# Autodesk Inventor assembly: 감속기어1
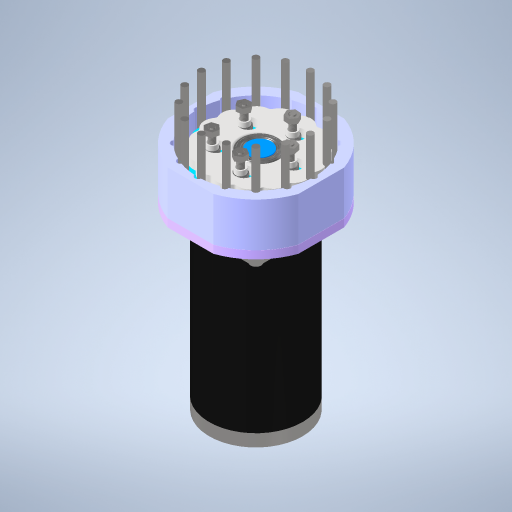
[picture p0: Inventor's stored thumbnail of the model, 512x512]
Saved by Autodesk Inventor 2023 (Build 270158000, 158)
## iProperties
Created: 2022-06-20
Part Number: 감속기어1
Document SubType Name: Assembly
Designer: user
Author: user
## Documents named in this file (19)
- C:\Users\user\Desktop\Baymax-main\설계\출력 부품\감속기어1.iam
- C:\Users\user\Desktop\Baymax-main\설계\범용 부품\베어링 6810.ipt
- C:\Users\user\Desktop\Baymax-main\설계\범용 부품\M4 16mm 십자나사.ipt
- C:\Users\user\Desktop\Baymax-main\설계\범용 부품\M4 너트.ipt
- C:\Users\user\Desktop\Baymax-main\설계\범용 부품\중형 모터 MB60080-2430 DC24V.ipt
- C:\Users\user\Desktop\Baymax-main\설계\출력 부품\감속기어1 - 기어 하우징.ipt
- C:\Users\user\Desktop\Baymax-main\설계\출력 부품\감속기어1 - 사이클로이드 기어.ipt
- C:\Users\user\Desktop\Baymax-main\설계\출력 부품\감속기어1 - 사이클로이드 회전축.ipt
- C:\Users\user\Desktop\Baymax-main\설계\범용 부품\M4 30mm 십자나사.ipt
- C:\Users\user\Desktop\Baymax-main\설계\출력 부품\감속기어1 - 축.ipt
- C:\Users\user\Desktop\Baymax-main\설계\범용 부품\베어링 6802.ipt
- C:\Users\user\Desktop\Baymax-main\설계\범용 부품\베어링 MR84ZZ.ipt
- C:\Users\user\Desktop\Baymax-main\설계\출력 부품\감속기어1 - 하우징 커버.ipt
- C:\Users\user\Desktop\Baymax-main\설계\범용 부품\4파이 20mm 핀.ipt
- C:\Users\user\Desktop\Baymax-main\설계\출력 부품\감속기어1 - 상단 편심축.ipt
- C:\Users\user\Desktop\Baymax-main\설계\출력 부품\감속기어1 - 4파이 4mm와셔.ipt
- C:\Users\user\Desktop\Baymax-main\설계\출력 부품\감속기어1 - 4파이 3mm와셔.ipt
- C:\Users\user\Desktop\Baymax-main\설계\출력 부품\감속기어1 - 회전축 상단.ipt
- C:\Users\user\Desktop\Baymax-main\설계\출력 부품\감속기어1 - 하우징 상단 커버.ipt
## Components (72 placed, 18 different names)
1. 베어링 6810:1 — 회전:5, 삽입:2
2. 중형 모터 MB60080-2430 DC24V:1 — 강체:1, 회전:7, 회전:8, 회전:9, 삽입:5, 회전:14
3. 감속기어1 - 기어 하우징:1 — 회전:1, 회전:2, 회전:3, 회전:4, 회전:5, 회전:13, 회전:15, 메이트:16
4. 감속기어1 - 사이클로이드 기어:1 — 삽입:4
5. 감속기어1 - 사이클로이드 회전축:1 — 강체:2, 강체:3, 회전:10, 회전:11, 회전:12, 삽입:2, 메이트:1, 메이트:2, 메이트:3, 메이트:4, 메이트:5, 메이트:6, 메이트:7, 메이트:8, 메이트:9, 메이트:10
6. M4 너트:1 — 회전:4
7. M4 너트:2 — 회전:3
8. M4 너트:3 — 회전:2
9. M4 너트:4 — 회전:1
10. M4 16mm 십자나사:1 — 회전:7
11. M4 16mm 십자나사:2 — 강체:1
12. M4 16mm 십자나사:3 — 회전:9
13. M4 16mm 십자나사:4 — 회전:8
14. M4 30mm 십자나사:1 — 회전:10
15. M4 30mm 십자나사:2 — 강체:2
16. M4 30mm 십자나사:3 — 강체:3
17. M4 30mm 십자나사:4 — 회전:12
18. M4 30mm 십자나사:5 — 회전:11
19. 감속기어1 - 축:1 — 삽입:3, 삽입:5, 회전:16
20. 베어링 6802:1 — 삽입:3, 삽입:4
21. 베어링 MR84ZZ:1 — 메이트:11
22. M4 너트:6 — 메이트:3, 메이트:4, 메이트:11
23. M4 너트:7 — 메이트:7, 메이트:8, 메이트:13
24. M4 너트:8 — 메이트:9, 메이트:10, 메이트:15
25. M4 너트:9 — 메이트:1, 메이트:2, 메이트:12
26. M4 너트:10 — 메이트:5, 메이트:6, 메이트:14
27. 베어링 MR84ZZ:2 — 메이트:15
28. 베어링 MR84ZZ:3 — 메이트:14
29. 베어링 MR84ZZ:4 — 메이트:12
30. 베어링 MR84ZZ:5 — 메이트:13, 강체:4
31. 감속기어1 - 하우징 커버:1 — 회전:13, 회전:14
32. 감속기어1 - 상단 편심축:1 — 회전:16, 삽입:7
33. 감속기어1 - 사이클로이드 기어:2
34. 베어링 6802:2 — 삽입:7
35. 감속기어1 - 회전축 상단:1 — 회전:19, 회전:20
36. 감속기어1 - 하우징 상단 커버:1 — 메이트:16
37. 4파이 20mm 핀:1 — 회전:15
38. 4파이 20mm 핀:2
39. 4파이 20mm 핀:3
40. 4파이 20mm 핀:4
41. 4파이 20mm 핀:5
42. 4파이 20mm 핀:6
43. 4파이 20mm 핀:7
44. 4파이 20mm 핀:8
45. 4파이 20mm 핀:9
46. 4파이 20mm 핀:10
47. 4파이 20mm 핀:11
48. 4파이 20mm 핀:12
49. 4파이 20mm 핀:13
50. 4파이 20mm 핀:14
51. 4파이 20mm 핀:15
52. 4파이 20mm 핀:16
53. 베어링 MR84ZZ:6 — 강체:4, 회전:18
54. 베어링 MR84ZZ:7 — 회전:17
55. 베어링 MR84ZZ:8
56. 베어링 MR84ZZ:9
57. 베어링 MR84ZZ:10
58. 감속기어1 - 4파이 4mm와셔:1 — 회전:17
59. 감속기어1 - 4파이 4mm와셔:2
60. 감속기어1 - 4파이 4mm와셔:3
61. 감속기어1 - 4파이 4mm와셔:4
62. 감속기어1 - 4파이 4mm와셔:5
63. 감속기어1 - 4파이 3mm와셔:1 — 회전:18
64. 감속기어1 - 4파이 3mm와셔:2
65. 감속기어1 - 4파이 3mm와셔:3
66. 감속기어1 - 4파이 3mm와셔:4
67. 감속기어1 - 4파이 3mm와셔:5 — 회전:19
68. M4 너트:11 — 회전:20
69. M4 너트:12
70. M4 너트:13
71. M4 너트:14
72. M4 너트:15
## Component patterns: (16 elements, first: 4파이 20mm 핀:1), (5 elements, first: 베어링 MR84ZZ:6), (5 elements, first: 감속기어1 - 4파이 4mm와셔:1), (5 elements, first: 감속기어1 - 4파이 3mm와셔:1), (5 elements, first: M4 너트:11)
## Relationships (45: RevoluteJoint 19, Mate 16, Insert 6, WeldJoint 4)
- 회전:1 [RevoluteJoint]: 감속기어1 - 기어 하우징:1 ↔ M4 너트:4
- 회전:2 [RevoluteJoint]: 감속기어1 - 기어 하우징:1 ↔ M4 너트:3
- 회전:3 [RevoluteJoint]: 감속기어1 - 기어 하우징:1 ↔ M4 너트:2
- 회전:4 [RevoluteJoint]: 감속기어1 - 기어 하우징:1 ↔ M4 너트:1
- 회전:5 [RevoluteJoint]: 베어링 6810:1 ↔ 감속기어1 - 기어 하우징:1
- 강체:1 [WeldJoint]: 중형 모터 MB60080-2430 DC24V:1 ↔ M4 16mm 십자나사:2
- 회전:7 [RevoluteJoint]: 중형 모터 MB60080-2430 DC24V:1 ↔ M4 16mm 십자나사:1
- 회전:8 [RevoluteJoint]: 중형 모터 MB60080-2430 DC24V:1 ↔ M4 16mm 십자나사:4
- 회전:9 [RevoluteJoint]: 중형 모터 MB60080-2430 DC24V:1 ↔ M4 16mm 십자나사:3
- 강체:2 [WeldJoint]: 감속기어1 - 사이클로이드 회전축:1 ↔ M4 30mm 십자나사:2
- 강체:3 [WeldJoint]: 감속기어1 - 사이클로이드 회전축:1 ↔ M4 30mm 십자나사:3
- 회전:10 [RevoluteJoint]: 감속기어1 - 사이클로이드 회전축:1 ↔ M4 30mm 십자나사:1
- 회전:11 [RevoluteJoint]: 감속기어1 - 사이클로이드 회전축:1 ↔ M4 30mm 십자나사:5
- 회전:12 [RevoluteJoint]: 감속기어1 - 사이클로이드 회전축:1 ↔ M4 30mm 십자나사:4
- 삽입:2 [Insert]: 베어링 6810:1 ↔ 감속기어1 - 사이클로이드 회전축:1
- 삽입:3 [Insert]: 감속기어1 - 축:1 ↔ 베어링 6802:1
- 삽입:4 [Insert]: 감속기어1 - 사이클로이드 기어:1 ↔ 베어링 6802:1
- 삽입:5 [Insert]: 중형 모터 MB60080-2430 DC24V:1 ↔ 감속기어1 - 축:1
- 메이트:1 [Mate]: 감속기어1 - 사이클로이드 회전축:1 ↔ M4 너트:9
- 메이트:2 [Mate]: 감속기어1 - 사이클로이드 회전축:1 ↔ M4 너트:9
- 메이트:3 [Mate]: 감속기어1 - 사이클로이드 회전축:1 ↔ M4 너트:6
- 메이트:4 [Mate]: 감속기어1 - 사이클로이드 회전축:1 ↔ M4 너트:6
- 메이트:5 [Mate]: 감속기어1 - 사이클로이드 회전축:1 ↔ M4 너트:10
- 메이트:6 [Mate]: 감속기어1 - 사이클로이드 회전축:1 ↔ M4 너트:10
- 메이트:7 [Mate]: 감속기어1 - 사이클로이드 회전축:1 ↔ M4 너트:7
- 메이트:8 [Mate]: 감속기어1 - 사이클로이드 회전축:1 ↔ M4 너트:7
- 메이트:9 [Mate]: 감속기어1 - 사이클로이드 회전축:1 ↔ M4 너트:8
- 메이트:10 [Mate]: 감속기어1 - 사이클로이드 회전축:1 ↔ M4 너트:8
- 메이트:11 [Mate]: 베어링 MR84ZZ:1 ↔ M4 너트:6
- 메이트:12 [Mate]: M4 너트:9 ↔ 베어링 MR84ZZ:4
- 메이트:13 [Mate]: M4 너트:7 ↔ 베어링 MR84ZZ:5
- 메이트:14 [Mate]: M4 너트:10 ↔ 베어링 MR84ZZ:3
- 메이트:15 [Mate]: M4 너트:8 ↔ 베어링 MR84ZZ:2
- 회전:13 [RevoluteJoint]: 감속기어1 - 기어 하우징:1 ↔ 감속기어1 - 하우징 커버:1
- 회전:14 [RevoluteJoint]: 중형 모터 MB60080-2430 DC24V:1 ↔ 감속기어1 - 하우징 커버:1
- 회전:15 [RevoluteJoint]: 감속기어1 - 기어 하우징:1 ↔ 4파이 20mm 핀:1
- 회전:16 [RevoluteJoint]: 감속기어1 - 축:1 ↔ 감속기어1 - 상단 편심축:1
- [Insert]: 감속기어1 - 사이클로이드 기어:2 ↔ 베어링 6802:2
- 삽입:7 [Insert]: 감속기어1 - 상단 편심축:1 ↔ 베어링 6802:2
- 강체:4 [WeldJoint] (4 mm): 베어링 MR84ZZ:5 ↔ 베어링 MR84ZZ:6
- 회전:17 [RevoluteJoint]: 베어링 MR84ZZ:7 ↔ 감속기어1 - 4파이 4mm와셔:1
- 회전:18 [RevoluteJoint]: 베어링 MR84ZZ:6 ↔ 감속기어1 - 4파이 3mm와셔:1
- 메이트:16 [Mate]: 감속기어1 - 기어 하우징:1 ↔ 감속기어1 - 하우징 상단 커버:1
- 회전:19 [RevoluteJoint]: 감속기어1 - 회전축 상단:1 ↔ 감속기어1 - 4파이 3mm와셔:5
- 회전:20 [RevoluteJoint]: 감속기어1 - 회전축 상단:1 ↔ M4 너트:11
## Named parameters: d72_d39 = 0 mm
